# Autodesk Inventor assembly: robot
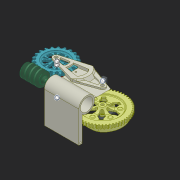
[picture p0: Inventor's stored thumbnail of the model, 180x180]
Saved by Autodesk Inventor 2020 (Build 240168000, 168)
## iProperties
Created: 2020-07-14
Part Number: robot
Document SubType Name: Assembly
Designer: alons
Author: alons
## Documents named in this file (11)
- C:\Users\alons\OneDrive\Documents\GitHub\Water-Strider-Robot\Striderbot\robot.iam
- C:\Users\alons\OneDrive\Documents\GitHub\Water-Strider-Robot\Striderbot\spur_gears_mesh_2\Design Accelerator\Spur Gear13.ipt
- C:\Users\alons\OneDrive\Documents\GitHub\Water-Strider-Robot\Striderbot\spur_gears_mesh_2\Design Accelerator\Spur Gear23.ipt
- C:\Users\alons\OneDrive\Documents\GitHub\Water-Strider-Robot\Striderbot\spur_gears_mesh_3\Design Accelerator\Spur Gear11.ipt
- C:\Users\alons\OneDrive\Documents\GitHub\Water-Strider-Robot\Striderbot\spur_gears_mesh_3\Design Accelerator\Spur Gear21.ipt
- C:\Users\alons\OneDrive\Documents\GitHub\Water-Strider-Robot\Striderbot\worm_gear_mesh_1\Design Accelerator\Worm Gear14.ipt
- C:\Users\alons\OneDrive\Documents\GitHub\Water-Strider-Robot\Striderbot\Crank_Rocker\Link_1.ipt
- C:\Users\alons\OneDrive\Documents\GitHub\Water-Strider-Robot\Striderbot\Crank_Rocker\Link_2.ipt
- C:\Users\alons\OneDrive\Documents\GitHub\Water-Strider-Robot\Striderbot\Crank_Rocker\Link_3.ipt
- C:\Users\alons\OneDrive\Documents\GitHub\Water-Strider-Robot\Striderbot\worm_gear_mesh_1\Design Accelerator\Worm14.ipt
- C:\Users\alons\OneDrive\Documents\GitHub\Water-Strider-Robot\Striderbot\top_frame.ipt
## Components (10 placed, 8 different names)
1. Spur Gear1:1 — Mate:1, Mate:2, Flush:1, Mate:3, Rotation:1, Mate:10, Mate:11
2. Spur Gear2:1 — Flush:1, Mate:3, Mate:4, Rotation:1, Flush:2, Mate:6
3. Spur Gear1:2 — Mate:5, Flush:2, Mate:6, Flush:3, Mate:7, Rotation:3, Mate:19
4. Spur Gear2:2 — Flush:3, Mate:7, Mate:8, Rotation:3, Mate:12, Mate:13, Mate:14
5. Worm Gear:1 — Mate:9, Mate:10, Mate:11, Rotation:4
6. Link_1:1 — Mate:12, Mate:13, Mate:14, Mate:15, Mate:16
7. Link_2:1 — Mate:15, Mate:16, Mate:17, Mate:18
8. Link_3:1 — Mate:17, Mate:18, Mate:19
9. Worm:1 — Mate:20, Flush:4, Mate:21, Rotation:4, Mate:22
10. top_frame:1 — Mate:22, Flush:5
## Relationships (30: Mate 22, Flush 5, RelateRotation 3)
- Mate:1 (-2 mm): Spur Gear1:1
- Mate:2: Spur Gear1:1
- Flush:1: Spur Gear1:1 ↔ Spur Gear2:1
- Mate:3 (6.3 mm): Spur Gear1:1 ↔ Spur Gear2:1
- Mate:4: Spur Gear2:1
- Rotation:1 [RelateRotation] (0.2812 ul): Spur Gear1:1 ↔ Spur Gear2:1
- Mate:5 (-5 mm): Spur Gear1:2
- Flush:2: Spur Gear2:1 ↔ Spur Gear1:2
- Mate:6: Spur Gear2:1 ↔ Spur Gear1:2
- Flush:3: Spur Gear1:2 ↔ Spur Gear2:2
- Mate:7 (8.45 mm): Spur Gear1:2 ↔ Spur Gear2:2
- Mate:8: Spur Gear2:2
- Rotation:3 [RelateRotation] (5.689 ul): Spur Gear1:2 ↔ Spur Gear2:2
- Mate:9: Worm Gear:1
- Mate:10: Spur Gear1:1 ↔ Worm Gear:1
- Mate:11: Spur Gear1:1 ↔ Worm Gear:1
- Mate:12: Spur Gear2:2 ↔ Link_1:1
- Mate:13: Spur Gear2:2 ↔ Link_1:1
- Mate:14 (2 mm): Spur Gear2:2 ↔ Link_1:1
- Mate:15: Link_1:1 ↔ Link_2:1
- Mate:16: Link_1:1 ↔ Link_2:1
- Mate:17: Link_2:1 ↔ Link_3:1
- Mate:18: Link_2:1 ↔ Link_3:1
- Mate:19: Spur Gear1:2 ↔ Link_3:1
- Mate:20 (-6.8 mm): Worm:1
- Flush:4: Worm:1
- Mate:21: Worm:1
- Rotation:4 [RelateRotation] (0.0455 ul): Worm Gear:1 ↔ Worm:1
- Mate:22: Worm:1 ↔ top_frame:1
- Flush:5: top_frame:1
